# Autodesk Inventor assembly: V3Cata
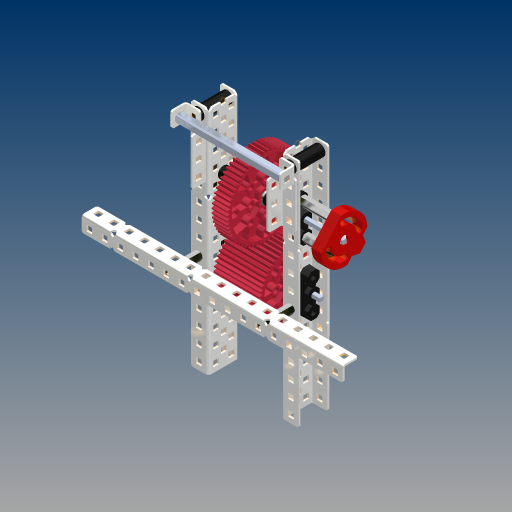
[picture p0: Inventor's stored thumbnail of the model, 512x512]
Saved by Autodesk Inventor 2023 (Build 270158000, 158)
## iProperties
Created: 2023-09-23
Part Number: V3Cata
Document SubType Name: Assembly
Designer: eddie
Author: eddie
## Documents named in this file (30)
- C:\Users\eddie\Documents\81208X-Over-Under-CAD\V3\V3Cata.iam
- C:\Users\eddie\Documents\81208X-Over-Under-CAD\VEX-CAD-Inventor-1.4.0\Structure\Angle\Aluminum\1x1\Alu Angle 1x1x17.ipt
- C:\Users\eddie\Documents\81208X-Over-Under-CAD\VEX-CAD-Inventor-1.4.0\Structure\Standoff\Standoff 1.00.ipt
- C:\Users\eddie\Documents\81208X-Over-Under-CAD\VEX-CAD-Inventor-1.4.0\Structure\Standoff.ipt
- C:\Users\eddie\Documents\81208X-Over-Under-CAD\VEX-CAD-Inventor-1.4.0\Structure\C Channel\Aluminum 1x2x1\Alu C 1x2x1x15.ipt
- C:\Users\eddie\Documents\81208X-Over-Under-CAD\VEX-CAD-Inventor-1.4.0\Structure\Angle\Aluminum\1x1\Alu Angle 1x1x3.ipt
- C:\Users\eddie\Documents\81208X-Over-Under-CAD\VEX-CAD-Inventor-1.4.0\Motion\Spacers\Spacer Nylon .375 OD\NSpacer .375 OD x .125.ipt
- C:\Users\eddie\Documents\81208X-Over-Under-CAD\VEX-CAD-Inventor-1.4.0\Motion\Spacers\Spacer Nylon .375 OD.ipt
- C:\Users\eddie\Documents\81208X-Over-Under-CAD\VEX-CAD-Inventor-1.4.0\Motion\Shaft HS\Shaft HS\Shaft HS 3.5 in.ipt
- C:\Users\eddie\Documents\81208X-Over-Under-CAD\VEX-CAD-Inventor-1.4.0\Motion\Shaft HS\Shaft HS.ipt
- C:\Users\eddie\Documents\81208X-Over-Under-CAD\VEX-CAD-Inventor-1.4.0\Structure\Angle\Aluminum\1x1\Alu Angle 1x1x1.ipt
- C:\Users\eddie\Documents\81208X-Over-Under-CAD\VEX-CAD-Inventor-1.4.0\Electronics\Sensors\Potentiometer.ipt
- C:\Users\eddie\Documents\81208X-Over-Under-CAD\Custom-parts\Bearing Flat with two holes.ipt
- C:\Users\eddie\Documents\81208X-Over-Under-CAD\VEX-CAD-Inventor-1.4.0\Motion\Shaft LS\Shaft LS.ipt
- C:\Users\eddie\Documents\81208X-Over-Under-CAD\VEX-CAD-Inventor-1.4.0\Motion\Shaft LS\Shaft LS\Shaft LS 4.0.ipt
- C:\Users\eddie\Documents\81208X-Over-Under-CAD\VEX-CAD-Inventor-1.4.0\Motion\Spacers\Spacer Nylon .375 OD\NSpacer .375 OD x .375.ipt
- C:\Users\eddie\Documents\81208X-Over-Under-CAD\VEX-CAD-Inventor-1.4.0\Motion\Spacers\Spacer Nylon .375 OD\NSpacer .375 OD x .500.ipt
- C:\Users\eddie\Documents\81208X-Over-Under-CAD\VEX-CAD-Inventor-1.4.0\Motion\Spacers\Spacer Nylon .500 OD\NSpacer White .500 OD x .125.ipt
- C:\Users\eddie\Documents\81208X-Over-Under-CAD\VEX-CAD-Inventor-1.4.0\Motion\Spacers\Spacer Nylon .500 OD.ipt
- C:\Users\eddie\Documents\81208X-Over-Under-CAD\Custom-parts\Shaft Collar.ipt
- C:\Users\eddie\Documents\81208X-Over-Under-CAD\VEX-CAD-Inventor-1.4.0\Motion\Spacers\Washer Steel\SWasher .375 OD x .031250.ipt
- C:\Users\eddie\Documents\81208X-Over-Under-CAD\VEX-CAD-Inventor-1.4.0\Motion\Spacers\Washer Steel.ipt
- C:\Users\eddie\Documents\81208X-Over-Under-CAD\Custom-parts\shaved-48-tooth-gear.iam
- C:\Users\eddie\Documents\81208X-Over-Under-CAD\VEX-CAD-Inventor-1.4.0\Motion\Gears\HS Gear.iam
- C:\Users\eddie\Documents\81208X-Over-Under-CAD\Custom-parts\shaved-48-tooth-gear.ipt
- C:\Users\eddie\Documents\81208X-Over-Under-CAD\VEX-CAD-Inventor-1.4.0\Structure\Angle\Aluminum\1x1\Alu Angle 1x1x5.ipt
- C:\Users\eddie\Documents\81208X-Over-Under-CAD\VEX-CAD-Inventor-1.4.0\Motion\Shaft LS\Bearing Flat.ipt
- C:\Users\eddie\Documents\81208X-Over-Under-CAD\VEX-CAD-Inventor-1.4.0\Motion\Shaft LS\Shaft LS\Shaft LS 3.0.ipt
- C:\Users\eddie\Documents\81208X-Over-Under-CAD\VEX-CAD-Inventor-1.4.0\Motion\Spacers\Spacer Nylon .375 OD\NSpacer .375 OD x .250.ipt
- C:\Users\eddie\Documents\81208X-Over-Under-CAD\VEX-CAD-Inventor-1.4.0\Motion\Gears\HS Gear\HS 60T Gear, Square.iam
## Components (51 placed, 21 different names)
1. Alu Angle 1x1x17:1 — Insert:1, Insert:2
2. Standoff 1.00:1 — Insert:1, Insert:3
3. Standoff 1.00:2 — Insert:2, Insert:4
4. Alu C 1x2x1x15:1 — Insert:3, Insert:5, Insert:8, Insert:12, Insert:15, Insert:16, Insert:17, Insert:23, Insert:24, Insert:36, Insert:38, Insert:40, Insert:51
5. Alu C 1x2x1x15:2 — Insert:4, Insert:6, Insert:7, Insert:18, Insert:21, Insert:35, Insert:37, Insert:42
6. Alu Angle 1x1x3:1 — Insert:5
7. Alu Angle 1x1x3:2 — Insert:6
8. NSpacer .375 OD x .125:1 — Insert:8, Insert:10
9. NSpacer .375 OD x .125:2 — Insert:7, Insert:9
10. Alu Angle 1x1x1:1 — Insert:10
11. Alu Angle 1x1x1:2 — Insert:9, Insert:11
12. Shaft HS 3.5 in:1 — Insert:11
13. NSpacer .375 OD x .125:3 — Insert:12, Insert:13
14. Standoff 1.00:3 — Insert:13, Insert:14
15. Potentiometer:1 — Insert:14
16. Bearing Flat with two holes:2 — Insert:15, Insert:16
17. Standoff 1.00:4 — Insert:17, Insert:20
18. Bearing Flat with two holes:3 — Insert:18, Insert:27
19. NSpacer .375 OD x .125:4 — Insert:20
20. NSpacer .375 OD x .375:5 — Insert:21, Insert:22
21. NSpacer .375 OD x .500:6 — Insert:22
22. NSpacer .375 OD x .375:7 — Insert:24
23. NSpacer .375 OD x .500:8 — Insert:23
24. Shaft LS 4.0:1 — Insert:27
25. Alu Angle 1x1x5:1 — Insert:35
26. Alu Angle 1x1x5:2 — Insert:36
27. Bearing Flat:1 — Insert:37, Insert:39
28. Bearing Flat:2 — Insert:38
29. Shaft LS 3.0:2 — Insert:39
30. NSpacer White .500 OD x .125:3 — Insert:40, Insert:41
31. NSpacer White .500 OD x .125:4 — Insert:42, Insert:43
32. Shaft Collar:3 — Insert:41, Insert:45
33. Shaft Collar:4 — Insert:43, Insert:44
34. shaved-48-tooth-gear:3 [sub-assembly] — Insert:47, Insert:48
35. SWasher .375 OD x .031250:3 — Insert:44
36. SWasher .375 OD x .031250:4 — Insert:45, Insert:47
37. shaved-48-tooth-gear:2 — Insert:48, Insert:49
38. shaved-48-tooth-gear:4 [sub-assembly] — Insert:49, Insert:50
39. SWasher .375 OD x .031250:5 — Insert:50
40. NSpacer .375 OD x .375:9 — Insert:51, Insert:52
41. SWasher .375 OD x .031250:6 — Insert:52, Insert:53
42. Shaft Collar:5 — Insert:53, Insert:54
43. NSpacer .375 OD x .250:10 — Insert:54, Insert:55
44. SWasher .375 OD x .031250:7 — Insert:56, Insert:57
45. SWasher .375 OD x .031250:8 — Insert:55, Insert:56
46. HS 60T Gear, Square:5 [sub-assembly] — Insert:57, Insert:58
47. SWasher .375 OD x .031250:9 — Insert:58, Insert:59
48. SWasher .375 OD x .031250:10 — Insert:59, Insert:60
49. SWasher .375 OD x .031250:11 — Insert:61, Insert:62
50. NSpacer .375 OD x .500:11 — Insert:60, Insert:61
51. NSpacer .375 OD x .375:12 — Insert:62
## Relationships (51: Insert 51)
- Insert:1: Alu Angle 1x1x17:1 ↔ Standoff 1.00:1
- Insert:2: Alu Angle 1x1x17:1 ↔ Standoff 1.00:2
- Insert:3: Standoff 1.00:1 ↔ Alu C 1x2x1x15:1
- Insert:4: Standoff 1.00:2 ↔ Alu C 1x2x1x15:2
- Insert:5: Alu C 1x2x1x15:1 ↔ Alu Angle 1x1x3:1
- Insert:6: Alu C 1x2x1x15:2 ↔ Alu Angle 1x1x3:2
- Insert:7: Alu C 1x2x1x15:2 ↔ NSpacer .375 OD x .125:2
- Insert:8: Alu C 1x2x1x15:1 ↔ NSpacer .375 OD x .125:1
- Insert:9: NSpacer .375 OD x .125:2 ↔ Alu Angle 1x1x1:2
- Insert:10: NSpacer .375 OD x .125:1 ↔ Alu Angle 1x1x1:1
- Insert:11: Alu Angle 1x1x1:2 ↔ Shaft HS 3.5 in:1
- Insert:12: Alu C 1x2x1x15:1 ↔ NSpacer .375 OD x .125:3
- Insert:13: NSpacer .375 OD x .125:3 ↔ Standoff 1.00:3
- Insert:14: Standoff 1.00:3 ↔ Potentiometer:1
- Insert:15: Alu C 1x2x1x15:1 ↔ Bearing Flat with two holes:2
- Insert:16: Alu C 1x2x1x15:1 ↔ Bearing Flat with two holes:2
- Insert:17: Alu C 1x2x1x15:1 ↔ Standoff 1.00:4
- Insert:18: Alu C 1x2x1x15:2 ↔ Bearing Flat with two holes:3
- Insert:20: Standoff 1.00:4 ↔ NSpacer .375 OD x .125:4
- Insert:21: Alu C 1x2x1x15:2 ↔ NSpacer .375 OD x .375:5
- Insert:22: NSpacer .375 OD x .375:5 ↔ NSpacer .375 OD x .500:6
- Insert:23: Alu C 1x2x1x15:1 ↔ NSpacer .375 OD x .500:8
- Insert:24: Alu C 1x2x1x15:1 ↔ NSpacer .375 OD x .375:7
- Insert:27: Bearing Flat with two holes:3 ↔ Shaft LS 4.0:1
- Insert:35: Alu C 1x2x1x15:2 ↔ Alu Angle 1x1x5:1
- Insert:36: Alu C 1x2x1x15:1 ↔ Alu Angle 1x1x5:2
- Insert:37: Alu C 1x2x1x15:2 ↔ Bearing Flat:1
- Insert:38: Alu C 1x2x1x15:1 ↔ Bearing Flat:2
- Insert:39: Bearing Flat:1 ↔ Shaft LS 3.0:2
- Insert:40: Alu C 1x2x1x15:1 ↔ NSpacer White .500 OD x .125:3
- Insert:41: NSpacer White .500 OD x .125:3 ↔ Shaft Collar:3
- Insert:42: Alu C 1x2x1x15:2 ↔ NSpacer White .500 OD x .125:4
- Insert:43: NSpacer White .500 OD x .125:4 ↔ Shaft Collar:4
- Insert:44: Shaft Collar:4 ↔ SWasher .375 OD x .031250:3
- Insert:45: Shaft Collar:3 ↔ SWasher .375 OD x .031250:4
- Insert:47: shaved-48-tooth-gear:3 ↔ SWasher .375 OD x .031250:4
- Insert:48: shaved-48-tooth-gear:3 ↔ shaved-48-tooth-gear:2
- Insert:49: shaved-48-tooth-gear:2 ↔ shaved-48-tooth-gear:4
- Insert:50: shaved-48-tooth-gear:4 ↔ SWasher .375 OD x .031250:5
- Insert:51: Alu C 1x2x1x15:1 ↔ NSpacer .375 OD x .375:9
- Insert:52: NSpacer .375 OD x .375:9 ↔ SWasher .375 OD x .031250:6
- Insert:53: SWasher .375 OD x .031250:6 ↔ Shaft Collar:5
- Insert:54: Shaft Collar:5 ↔ NSpacer .375 OD x .250:10
- Insert:55: NSpacer .375 OD x .250:10 ↔ SWasher .375 OD x .031250:8
- Insert:56: SWasher .375 OD x .031250:7 ↔ SWasher .375 OD x .031250:8
- Insert:57: SWasher .375 OD x .031250:7 ↔ HS 60T Gear, Square:5
- Insert:58: HS 60T Gear, Square:5 ↔ SWasher .375 OD x .031250:9
- Insert:59: SWasher .375 OD x .031250:9 ↔ SWasher .375 OD x .031250:10
- Insert:60: SWasher .375 OD x .031250:10 ↔ NSpacer .375 OD x .500:11
- Insert:61: SWasher .375 OD x .031250:11 ↔ NSpacer .375 OD x .500:11
- Insert:62: SWasher .375 OD x .031250:11 ↔ NSpacer .375 OD x .375:12
